# Autodesk Inventor assembly: Assembly_Cube_Objective_Holder_v3
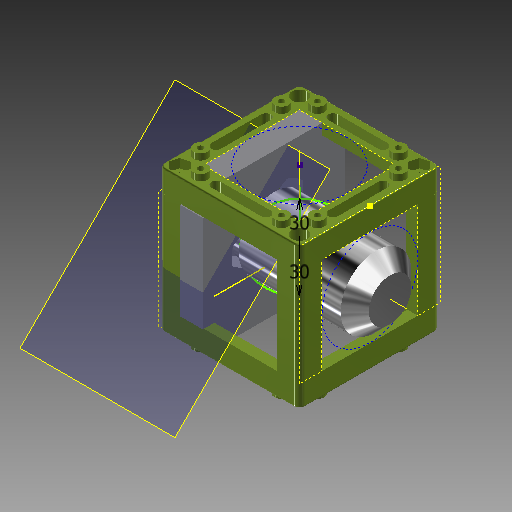
[picture p0: Inventor's stored thumbnail of the model, 512x512]
Saved by Autodesk Inventor 2019 (Build 230136000, 136)
## iProperties
Created: 2018-06-11
Part Number: Assembly_Cube_Objective_Holder_v3
Material: Generisch
Document SubType Name: Assembly
Designer: diederichbenedict
Mass: 58.1372 g
Surface Area: 256.675 cm^2
Volume: 50.1049 cm^3
Density: 1.16031 g/cm^3
Author: diederichbenedict
## Documents named in this file (4)
- C:\Users\marsikovabarbora\Dropbox\UC2\02_CAD\INVENTOR\uc2_v3\Assembly_Cube_Objective_Holder_v3.iam
- C:\Users\marsikovabarbora\Dropbox\UC2\02_CAD\INVENTOR\uc2_v3\00_Microscope_Objective_Lens10x.ipt
- C:\Users\marsikovabarbora\Dropbox\UC2\02_CAD\INVENTOR\uc2_v3\Assembly_Cube_empty_IM_v3.iam
- C:\Users\marsikovabarbora\Dropbox\UC2\02_CAD\INVENTOR\uc2_v3\20_Cube_Insert_Lens_holder_RMS_63x.ipt
## Components (3 placed, 3 different names)
1. 00_Microscope_Objective_Lens10x:1 — Mate:1, Mate:4
2. Assembly_Cube_empty_IM_v3:2 [sub-assembly] — Mate:1, Mate:2, Mate:3, Angle:1
3. 20_Cube_Insert_Lens_holder_RMS_63x:1 — Mate:2, Mate:3, Angle:1, Mate:4
## Relationships (5: Mate 4, Angle 1)
- Mate:1: 00_Microscope_Objective_Lens10x:1 ↔ Assembly_Cube_empty_IM_v3:2
- Mate:2: Assembly_Cube_empty_IM_v3:2 ↔ 20_Cube_Insert_Lens_holder_RMS_63x:1
- Mate:3: Assembly_Cube_empty_IM_v3:2 ↔ 20_Cube_Insert_Lens_holder_RMS_63x:1
- Angle:1 (0 deg): Assembly_Cube_empty_IM_v3:2 ↔ 20_Cube_Insert_Lens_holder_RMS_63x:1
- Mate:4: 00_Microscope_Objective_Lens10x:1 ↔ 20_Cube_Insert_Lens_holder_RMS_63x:1
